# Autodesk Inventor assembly: SwitchOnTNutHolderRight
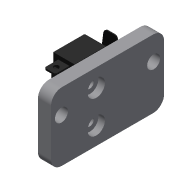
[picture p0: Inventor's stored thumbnail of the model, 180x180]
Saved by Autodesk Inventor 2018 (Build 220112000, 112)
## iProperties
Created: 2018-12-20
Part Number: SwitchOnTNutHolderRight
Document SubType Name: Assembly
Designer: ball
Author: ball
## Documents named in this file (3)
- C:\FTC\FTC8863CAD\2018Robot\SwitchOnTNutHolderRight.iam
- C:\FTC\FTC8863CAD\2018Robot\SwitchHolderTNutRight.ipt
- C:\FTC\FTC8863CAD\Actobotics\605 parts\605630.ipt
## Components (2 placed, 2 different names)
1. SwitchHolderTNutRight:1 — Mate:1, Mate:2, Mate:3
2. 605630:1 — Mate:1, Mate:2, Mate:3
## Relationships (3: Mate 3)
- Mate:1: SwitchHolderTNutRight:1 ↔ 605630:1
- Mate:2: SwitchHolderTNutRight:1 ↔ 605630:1
- Mate:3: SwitchHolderTNutRight:1 ↔ 605630:1
